# Autodesk Inventor assembly: Pancake_Pneumatic_Cylinder_217-2778 (3)
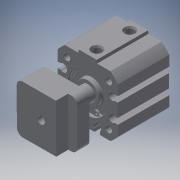
[picture p0: Inventor's stored thumbnail of the model, 180x180]
Saved by Autodesk Inventor 2019.4 (Build 234330000, 330)
## iProperties
Created: 2014-08-06
Part Number: Pancake_Pneumatic_Cylinder_217-2778 (3)
Description: STEP AP203
Document SubType Name: Assembly
Designer: mavericks
Sending System: SolidWorks 2014
Preprocessor: SwSTEP 2.0
Title: 217-2778-001 Rev2.STEP
Revision Number: ANY
## Documents named in this file (5)
- T:\EIT\2020 Infinite Recharge\2020 ROBOT\COMMON PARTS\AIR CYLINDERS\Pancake_Pneumatic_Cylinder_217-2778 (3).iam
- T:\EIT\2020 Infinite Recharge\2020 ROBOT\COMMON PARTS\AIR CYLINDERS\217-2778-NCQ8A075-050M_NCQ8 Tube_075A.ipt
- T:\EIT\2020 Infinite Recharge\2020 ROBOT\COMMON PARTS\AIR CYLINDERS\217-2778-NCQ8A075-050M_NCQ8 Rod_075M.ipt
- T:\EIT\2020 Infinite Recharge\2020 ROBOT\COMMON PARTS\AIR CYLINDERS\217-2778-NCQ8A075-050M_Snap Ring_075.ipt
- T:\EIT\2020 Infinite Recharge\2020 ROBOT\LIFT\LM-GB\LM-GB-018.ipt
## Components (4 placed, 4 different names)
1. 217-2778-NCQ8A075-050M_NCQ8 Tube_075A_1 — Insert:1
2. 217-2778-NCQ8A075-050M_NCQ8 Rod_075M_2 — Insert:1, Insert:2
3. 217-2778-NCQ8A075-050M_Snap Ring_075_3
4. LM-GB-018:1 — Insert:2
## Relationships (2: Insert 2)
- Insert:1: 217-2778-NCQ8A075-050M_NCQ8 Tube_075A_1 ↔ 217-2778-NCQ8A075-050M_NCQ8 Rod_075M_2
- Insert:2: 217-2778-NCQ8A075-050M_NCQ8 Rod_075M_2 ↔ LM-GB-018:1
